# Autodesk Inventor assembly: SAFRS-A-0012
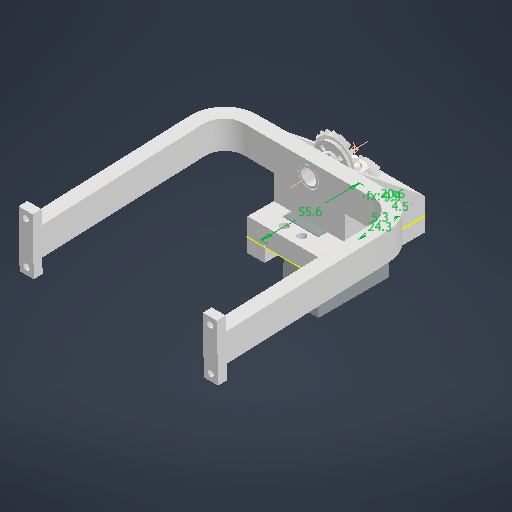
[picture p0: Inventor's stored thumbnail of the model, 512x512]
Saved by Autodesk Inventor 2026.2 (Build 302298000, 298)
## iProperties
Created: 2025-11-28
Part Number: SAFRS-A-0012
Document SubType Name: Assembly
Designer: jaewook
Author: jaewook
Title: Roll Support Front v2 Assembly
## Documents named in this file (6)
- C:\Users\jk000\OneDrive\Desktop\git\SAFRS\mechanical\inventor\02__subassemblies\roll_support_front_v2.iam
- C:\Users\jk000\OneDrive\Desktop\git\SAFRS\mechanical\inventor\01_parts\solid_7.ipt
- C:\Users\jk000\OneDrive\Desktop\git\SAFRS\mechanical\inventor\02__subassemblies\bevel_gear_pair_2.iam
- C:\Users\jk000\OneDrive\Desktop\git\SAFRS\mechanical\inventor\01_parts\motor_clamp.ipt
- C:\Users\jk000\OneDrive\Desktop\git\SAFRS\mechanical\inventor\01_parts\connector.ipt
- C:\Users\jk000\OneDrive\Desktop\git\SAFRS\mechanical\inventor\01_parts\servo_ds35mg_180.ipt
## Components (5 placed, 5 different names)
1. solid_7:2 — 메이트:3, 메이트:4, 메이트:7, 메이트:8
2. 베벨 기어:1 [sub-assembly] — 메이트:1, 메이트:2, 메이트:5, 메이트:6
3. motor_clamp:2 — 메이트:1, 메이트:2, 메이트:3, 메이트:4
4. connector:1 — 메이트:5, 메이트:6
5. servo_ds35mg_180:1 — 메이트:7, 메이트:8
## Relationships (8: Mate 8)
- 메이트:1 [Mate]: 베벨 기어:1 ↔ motor_clamp:2
- 메이트:2 [Mate]: 베벨 기어:1 ↔ motor_clamp:2
- 메이트:3 [Mate]: solid_7:2 ↔ motor_clamp:2
- 메이트:4 [Mate]: solid_7:2 ↔ motor_clamp:2
- 메이트:5 [Mate]: 베벨 기어:1 ↔ connector:1
- 메이트:6 [Mate]: 베벨 기어:1 ↔ connector:1
- 메이트:7 [Mate]: solid_7:2 ↔ servo_ds35mg_180:1
- 메이트:8 [Mate]: solid_7:2 ↔ servo_ds35mg_180:1
